# Autodesk Inventor assembly: Assembly_center_unit
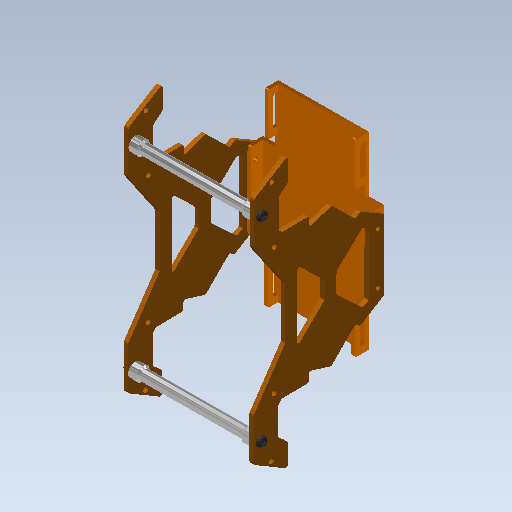
[picture p0: Inventor's stored thumbnail of the model, 512x512]
Saved by Autodesk Inventor 2020 (Build 240168000, 168)
## iProperties
Created: 2019-09-25
Part Number: Assembly_center_unit
Document SubType Name: Assembly
Designer: maste
Author: maste
## Documents named in this file (8)
- C:\Users\maste\Documents\GitHub\autobot\robot_model\Assembly_center_unit.iam
- C:\Users\maste\Documents\GitHub\autobot\robot_model\RCT-H112_stick_battery_plate.ipt
- C:\Users\maste\Documents\GitHub\autobot\robot_model\RCT-H001_Al_side_plate.ipt
- C:\Users\maste\Documents\GitHub\autobot\robot_model\RCT-H010_Al_side_plate_post.ipt
- C:\Users\maste\Documents\GitHub\autobot\robot_model\Assembly_center_unit\Design Accelerator\assembly_center_unit_BC_01.iam
- C:\Users\maste\Documents\GitHub\autobot\robot_model\Assembly_center_unit\Design Accelerator\Assembly_center_unit_BC_02.iam
- C:\Users\maste\Documents\GitHub\autobot\robot_model\Assembly_center_unit\Design Accelerator\Assembly_center_unit_BC_03.iam
- C:\Users\maste\Documents\GitHub\autobot\robot_model\Assembly_center_unit\Design Accelerator\Assembly_center_unit_BC_04.iam
## Components (9 placed, 4 different names)
1. RCT-H112_stick_battery_plate:1 — Mate:1, Mate:2, Mate:3, Mate:4, Mate:5, Mate:6
2. RCT-H001_Al_side_plate:1 — Mate:1, Mate:2, Mate:3, Mate:7, Mate:8, Mate:9, Mate:10, Mate:11, Mate:12, Mate:13, Mate:14
3. RCT-H001_Al_side_plate:2 — Mate:4, Mate:5, Mate:6, Mate:15, Mate:16, Mate:17, Mate:18
4. RCT-H010_Al_side_plate_post:1 — Mate:7, Mate:8
5. RCT-H010_Al_side_plate_post:2 — Mate:9, Mate:10
6. Bolted Connection:1 [sub-assembly] — Mate:11, Mate:12
7. Bolted Connection:2 [sub-assembly] — Mate:13, Mate:14
8. Bolted Connection:3 [sub-assembly] — Mate:15, Mate:16
9. Bolted Connection:4 [sub-assembly] — Mate:17, Mate:18
## Relationships (18: Mate 18)
- Mate:1: RCT-H112_stick_battery_plate:1 ↔ RCT-H001_Al_side_plate:1
- Mate:2: RCT-H112_stick_battery_plate:1 ↔ RCT-H001_Al_side_plate:1
- Mate:3: RCT-H112_stick_battery_plate:1 ↔ RCT-H001_Al_side_plate:1
- Mate:4: RCT-H112_stick_battery_plate:1 ↔ RCT-H001_Al_side_plate:2
- Mate:5: RCT-H112_stick_battery_plate:1 ↔ RCT-H001_Al_side_plate:2
- Mate:6: RCT-H112_stick_battery_plate:1 ↔ RCT-H001_Al_side_plate:2
- Mate:7: RCT-H001_Al_side_plate:1 ↔ RCT-H010_Al_side_plate_post:1
- Mate:8: RCT-H001_Al_side_plate:1 ↔ RCT-H010_Al_side_plate_post:1
- Mate:9: RCT-H001_Al_side_plate:1 ↔ RCT-H010_Al_side_plate_post:2
- Mate:10: RCT-H001_Al_side_plate:1 ↔ RCT-H010_Al_side_plate_post:2
- Mate:11: RCT-H001_Al_side_plate:1 ↔ Bolted Connection:1
- Mate:12: RCT-H001_Al_side_plate:1 ↔ Bolted Connection:1
- Mate:13: RCT-H001_Al_side_plate:1 ↔ Bolted Connection:2
- Mate:14: RCT-H001_Al_side_plate:1 ↔ Bolted Connection:2
- Mate:15: RCT-H001_Al_side_plate:2 ↔ Bolted Connection:3
- Mate:16: RCT-H001_Al_side_plate:2 ↔ Bolted Connection:3
- Mate:17: RCT-H001_Al_side_plate:2 ↔ Bolted Connection:4
- Mate:18: RCT-H001_Al_side_plate:2 ↔ Bolted Connection:4
